# Autodesk Inventor assembly: CNC2
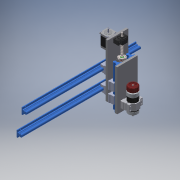
[picture p0: Inventor's stored thumbnail of the model, 180x180]
Saved by Autodesk Inventor 2018 (Build 220112000, 112)
## iProperties
Created: 2018-10-11
Part Number: CNC2
Material: Genérico
Document SubType Name: Assembly
Designer: Usuario
Author: Usuario
## Documents named in this file (14)
- C:\Users\Usuario\Documents\OpenCNC\MONTAGEM\CNC2.iam
- C:\Users\Usuario\Documents\OpenCNC\COMPONENTES_MECANICOS\BLOCOS_GUIAS_LINEARES\SBR16UU.ipt
- C:\Users\Usuario\Documents\OpenCNC\MONTAGEM\BLOCO_SUPORTE_EIXO_Z.ipt
- C:\Users\Usuario\Documents\OpenCNC\BAIXADOS\spindle-bldc-500w-1.snapshot.1\SPINDLE_500WSpindle.iam
- C:\Users\Usuario\Documents\OpenCNC\BAIXADOS\spindle-bracket-1.snapshot.2\SUPORTE_SPINDLESpindle Bracket.ipt
- C:\Users\Usuario\Documents\OpenCNC\MONTAGEM\CNC1\BLOCO_SUPORTE_SPINDLE.ipt
- C:\Users\Usuario\Documents\OpenCNC\BAIXADOS\sfu1204-300-with-nut-1.snapshot.3\CASTANHA_FUSO_SFU1204SFU1204-3.ipt
- C:\Users\Usuario\Documents\OpenCNC\BAIXADOS\stepper motor NEMA 23 57x76.ipt
- C:\Users\Usuario\Documents\OpenCNC\BAIXADOS\bearing-support-unit-1.snapshot.1\BK12BK12.ipt
- C:\Users\Usuario\Documents\OpenCNC\BAIXADOS\bearing-support-unit-1.snapshot.1\BF12.ipt
- C:\Users\Usuario\Documents\OpenCNC\BAIXADOS\sfu1204-300-with-nut-1.snapshot.3\FUSO_SFU1204SFU1204-300.ipt
- C:\Users\Usuario\Documents\OpenCNC\COMPONENTES_MECANICOS\GUIAS_LINEARES\SBR16_200MM.ipt
- C:\Users\Usuario\Documents\OpenCNC\COMPONENTES_MECANICOS\GUIAS_LINEARES\SBR16_EIXO_X_1.ipt
- C:\Users\Usuario\Documents\OpenCNC\COMPONENTES_MECANICOS\GUIAS_LINEARES\SBR16_EIXO_X_2.ipt
## Components (21 placed, 13 different names)
1. SBR16UU:1 — Coincidência:22, Alinhamento:36, Alinhamento:38, Alinhamento:39, Coincidência:25
2. SBR16UU:2 — Coincidência:21, Alinhamento:36, Alinhamento:40
3. SBR16UU:3 — Coincidência:23, Alinhamento:37, Alinhamento:38, Coincidência:26
4. SBR16UU:4 — Coincidência:24, Alinhamento:37, Alinhamento:41
5. BLOCO_SUPORTE_EIXO_Z:1 — Coincidência:21, Coincidência:22, Coincidência:23, Coincidência:24, Alinhamento:39, Alinhamento:40, Alinhamento:41
6. SPINDLE_500WSpindle:1 [sub-assembly]
7. SUPORTE_SPINDLESpindle Bracket:1
8. BLOCO_SUPORTE_SPINDLE:1
9. CASTANHA_FUSO_SFU1204SFU1204-3:1
10. stepper motor NEMA 23 57x76:1
11. BK12BK12:1
12. BF12:1
13. FUSO_SFU1204SFU1204-300:1
14. SBR16UU:5
15. SBR16UU:6
16. SBR16UU:7
17. SBR16UU:8
18. SBR16_200MM:1
19. SBR16_200MM:2
20. SBR16_EIXO_X_1:1 — Coincidência:25
21. SBR16_EIXO_X_2:1 — Coincidência:26
## Relationships (48: Flush 27, Mate 21)
- [Mate]: SUPORTE_SPINDLESpindle Bracket:1 ↔ BLOCO_SUPORTE_SPINDLE:1
- [Flush] (25 mm): SUPORTE_SPINDLESpindle Bracket:1 ↔ BLOCO_SUPORTE_SPINDLE:1
- [Flush] (18 mm): SUPORTE_SPINDLESpindle Bracket:1 ↔ BLOCO_SUPORTE_SPINDLE:1
- [Mate]: SPINDLE_500WSpindle:1 ↔ SUPORTE_SPINDLESpindle Bracket:1
- [Flush] (-25 mm): SPINDLE_500WSpindle:1 ↔ SUPORTE_SPINDLESpindle Bracket:1
- [Mate]: BLOCO_SUPORTE_EIXO_Z:1 ↔ BK12BK12:1
- [Mate]: BK12BK12:1 ↔ FUSO_SFU1204SFU1204-300:1
- [Flush] (18.31 mm): BK12BK12:1 ↔ FUSO_SFU1204SFU1204-300:1
- [Mate]: BF12:1 ↔ FUSO_SFU1204SFU1204-300:1
- [Flush] (-1.5 mm): BF12:1 ↔ FUSO_SFU1204SFU1204-300:1
- [Flush]: BK12BK12:1 ↔ BF12:1
- [Mate]: CASTANHA_FUSO_SFU1204SFU1204-3:1 ↔ FUSO_SFU1204SFU1204-300:1
- [Flush]: SBR16UU:5 ↔ SBR16UU:6
- [Flush]: SBR16UU:7 ↔ SBR16UU:8
- [Flush]: SBR16UU:5 ↔ SBR16UU:7
- [Flush]: SBR16UU:6 ↔ SBR16UU:8
- [Flush]: SBR16UU:6 ↔ SBR16UU:8
- [Flush]: SBR16UU:5 ↔ SBR16UU:6
- [Flush]: SBR16UU:7 ↔ SBR16UU:8
- [Mate] (23 mm): SBR16UU:5 ↔ SBR16UU:7
- [Mate] (35 mm): SBR16UU:5 ↔ SBR16UU:6
- [Mate]: BLOCO_SUPORTE_EIXO_Z:1 ↔ SBR16UU:5
- [Flush]: BLOCO_SUPORTE_EIXO_Z:1 ↔ SBR16UU:8
- [Mate]: SBR16UU:5 ↔ SBR16_200MM:1
- [Mate]: BLOCO_SUPORTE_SPINDLE:1 ↔ SBR16_200MM:1
- [Mate]: SBR16UU:6 ↔ SBR16_200MM:2
- [Mate]: BLOCO_SUPORTE_SPINDLE:1 ↔ SBR16_200MM:2
- [Flush]: BLOCO_SUPORTE_SPINDLE:1 ↔ SBR16_200MM:1
- [Flush]: BLOCO_SUPORTE_SPINDLE:1 ↔ SBR16_200MM:2
- [Flush] (-2.5 mm): BLOCO_SUPORTE_SPINDLE:1 ↔ SBR16_200MM:1
- [Flush]: BLOCO_SUPORTE_EIXO_Z:1 ↔ SBR16UU:5
- [Mate]: BLOCO_SUPORTE_SPINDLE:1 ↔ CASTANHA_FUSO_SFU1204SFU1204-3:1
- [Flush] (46.627 mm): BLOCO_SUPORTE_EIXO_Z:1 ↔ BF12:1
- [Flush] (32.5 mm): BLOCO_SUPORTE_EIXO_Z:1 ↔ BK12BK12:1
- [Mate]: BLOCO_SUPORTE_EIXO_Z:1 ↔ stepper motor NEMA 23 57x76:1
- [Flush]: stepper motor NEMA 23 57x76:1 ↔ BK12BK12:1
- Coincidência:21 [Mate]: SBR16UU:2 ↔ BLOCO_SUPORTE_EIXO_Z:1
- Coincidência:22 [Mate]: SBR16UU:1 ↔ BLOCO_SUPORTE_EIXO_Z:1
- Coincidência:23 [Mate]: SBR16UU:3 ↔ BLOCO_SUPORTE_EIXO_Z:1
- Coincidência:24 [Mate]: SBR16UU:4 ↔ BLOCO_SUPORTE_EIXO_Z:1
- Alinhamento:36 [Flush]: SBR16UU:1 ↔ SBR16UU:2
- Alinhamento:37 [Flush]: SBR16UU:3 ↔ SBR16UU:4
- Alinhamento:38 [Flush]: SBR16UU:1 ↔ SBR16UU:3
- Alinhamento:39 [Flush]: SBR16UU:1 ↔ BLOCO_SUPORTE_EIXO_Z:1
- Alinhamento:40 [Flush]: SBR16UU:2 ↔ BLOCO_SUPORTE_EIXO_Z:1
- Alinhamento:41 [Flush]: SBR16UU:4 ↔ BLOCO_SUPORTE_EIXO_Z:1
- Coincidência:25 [Mate]: SBR16UU:1 ↔ SBR16_EIXO_X_1:1
- Coincidência:26 [Mate]: SBR16UU:3 ↔ SBR16_EIXO_X_2:1
